# Autodesk Inventor assembly: Tea Steeping mechanism
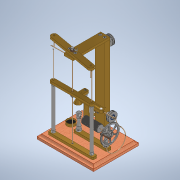
[picture p0: Inventor's stored thumbnail of the model, 180x180]
Saved by Autodesk Inventor 2021.1 (Build 251245010, 245A)
## iProperties
Created: 2025-09-16
Part Number: Tea Steeping mechanism
Document SubType Name: Assembly
Designer: SD
Mass: 7578.53 g
Surface Area: 3751.61 cm^2
Volume: 1764.11 cm^3
Density: 4.29596 g/cm^3
Project: Automatic Tea Steeping mechanism
BOM-Mass: 7.57853
BOM-Area: 0.375
Author: SD
Title: Automatic Tea Steeping mechanism
## Documents named in this file (8)
- S:\Future Scope 1\WIP\Client Category\Tom\02 Progressive Work\Automatic Tea Steeping mechanism.iam
- S:\Future Scope 1\WIP\Client Category\Tom\02 Progressive Work\Wooden Base.ipt
- S:\Future Scope 1\WIP\Client Category\Tom\02 Progressive Work\Main Piller And Support.iam
- S:\Future Scope 1\WIP\Client Category\Tom\02 Progressive Work\Upper Static Arms.iam
- S:\Future Scope 1\WIP\Client Category\Tom\02 Progressive Work\Lower Static Arms.iam
- S:\Future Scope 1\WIP\Client Category\Tom\02 Progressive Work\Rotating Assembly.iam
- S:\Future Scope 1\WIP\Client Category\Tom\02 Progressive Work\Wheel And Drum.iam
- S:\Future Scope 1\WIP\Client Category\Tom\02 Progressive Work\Steeping Complete Notification Contraption.iam
## Components (7 placed, 7 different names)
1. Wooden Base:1 — Mate:1, Mate:2, Mate:3, Mate:6, Mate:7, Mate:8, Mate:11, Mate:12, Mate:13, Mate:17, Mate:18, Angle:3
2. Main Piller And Support:1 [sub-assembly] — Mate:1, Mate:2, Mate:3, Mate:4, Angle:1, Mate:5, Mate:10
3. Upper Static Arms:1 [sub-assembly] — Mate:4, Angle:1, Mate:5, Mate:9
4. Lower Static Arms:1 [sub-assembly] — Mate:6, Mate:7, Mate:8, Angle:2
5. Rotating Assembly:1 [sub-assembly] — Mate:9, Mate:10, Angle:2
6. Wheel And Drum:1 [sub-assembly] — Mate:11, Mate:12, Mate:13
7. Steeping Complete Notification Contraption:1 [sub-assembly] — Mate:17, Mate:18, Angle:3
## Relationships (18: Mate 15, Angle 3)
- Mate:1: Wooden Base:1 ↔ Main Piller And Support:1
- Mate:2: Wooden Base:1 ↔ Main Piller And Support:1
- Mate:3: Wooden Base:1 ↔ Main Piller And Support:1
- Mate:4: Main Piller And Support:1 ↔ Upper Static Arms:1
- Angle:1 (-10 deg): Main Piller And Support:1 ↔ Upper Static Arms:1
- Mate:5: Main Piller And Support:1 ↔ Upper Static Arms:1
- Mate:6: Wooden Base:1 ↔ Lower Static Arms:1
- Mate:7: Wooden Base:1 ↔ Lower Static Arms:1
- Mate:8: Wooden Base:1 ↔ Lower Static Arms:1
- Mate:9: Upper Static Arms:1 ↔ Rotating Assembly:1
- Mate:10 (2 mm): Main Piller And Support:1 ↔ Rotating Assembly:1
- Angle:2 (0 deg): Lower Static Arms:1 ↔ Rotating Assembly:1
- Mate:11: Wooden Base:1 ↔ Wheel And Drum:1
- Mate:12: Wooden Base:1 ↔ Wheel And Drum:1
- Mate:13: Wooden Base:1 ↔ Wheel And Drum:1
- Mate:17: Wooden Base:1 ↔ Steeping Complete Notification Contraption:1
- Mate:18: Wooden Base:1 ↔ Steeping Complete Notification Contraption:1
- Angle:3 (180 deg): Wooden Base:1 ↔ Steeping Complete Notification Contraption:1
